# Autodesk Inventor assembly: Frank
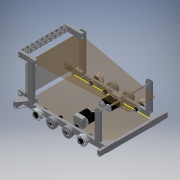
[picture p0: Inventor's stored thumbnail of the model, 180x180]
Saved by Autodesk Inventor 2018 (Build 220112000, 112)
## iProperties
Created: 2018-09-06
Part Number: Frank
Document SubType Name: Assembly
Designer: baoan
Author: baoan
## Documents named in this file (7)
- C:\Users\baoan\Documents\Inventor\Bunnybots\Frank.iam
- C:\Users\baoan\Documents\Inventor\Bunnybots\Drivetrain\Drivetrain.iam
- C:\Users\baoan\Documents\Inventor\Bunnybots\Electrical_board\Belly_pan.ipt
- C:\Users\baoan\Documents\Inventor\Bunnybots\Intake&Outake\Intake&Outake.iam
- C:\Users\baoan\Documents\Inventor\Bunnybots\Intake&Outake\Outtake_vertical_frame.ipt
- C:\Users\baoan\Documents\Inventor\Bunnybots\Intake&Outake\Ramp.ipt
- C:\Users\baoan\Documents\Inventor\Bunnybots\Intake&Outake\Outtake_churro.ipt
## Components (7 placed, 6 different names)
1. Drivetrain:1 [sub-assembly] — Mate:1, Mate:2, Mate:3, Mate:4, Flush:1, Mate:5, Mate:6, Flush:2, Mate:7, Mate:8, Flush:3, Mate:9
2. Belly_pan:1 — Mate:1, Mate:2, Mate:3
3. Intake&Outake:1 [sub-assembly] — Mate:4, Flush:1, Mate:5, Mate:12, Mate:13
4. Outtake_vertical_frame:1 — Mate:6, Flush:2, Mate:7, Mate:10, Mate:11
5. Outtake_vertical_frame:2 — Mate:8, Flush:3, Mate:9
6. Ramp:1 — Mate:12, Mate:13, Mate:14
7. Outtake_churro:1 — Mate:10, Mate:11, Mate:14
## Relationships (17: Mate 14, Flush 3)
- Mate:1: Drivetrain:1 ↔ Belly_pan:1
- Mate:2: Drivetrain:1 ↔ Belly_pan:1
- Mate:3: Drivetrain:1 ↔ Belly_pan:1
- Mate:4: Drivetrain:1 ↔ Intake&Outake:1
- Flush:1: Drivetrain:1 ↔ Intake&Outake:1
- Mate:5: Drivetrain:1 ↔ Intake&Outake:1
- Mate:6: Drivetrain:1 ↔ Outtake_vertical_frame:1
- Flush:2: Drivetrain:1 ↔ Outtake_vertical_frame:1
- Mate:7: Drivetrain:1 ↔ Outtake_vertical_frame:1
- Mate:8: Drivetrain:1 ↔ Outtake_vertical_frame:2
- Flush:3: Drivetrain:1 ↔ Outtake_vertical_frame:2
- Mate:9: Drivetrain:1 ↔ Outtake_vertical_frame:2
- Mate:10: Outtake_vertical_frame:1 ↔ Outtake_churro:1
- Mate:11: Outtake_vertical_frame:1 ↔ Outtake_churro:1
- Mate:12: Intake&Outake:1 ↔ Ramp:1
- Mate:13: Intake&Outake:1 ↔ Ramp:1
- Mate:14: Ramp:1 ↔ Outtake_churro:1
